# Autodesk Inventor assembly: buildplate
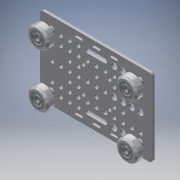
[picture p0: Inventor's stored thumbnail of the model, 180x180]
Saved by Autodesk Inventor 2016 (Build 200138000, 138)
## iProperties
Created: 2016-03-19
Part Number: buildplate
Document SubType Name: Assembly
Designer: Solomon
Author: Solomon
## Documents named in this file (4)
- C:\Users\Solomon\Documents\Inventor\SLA MK I\buildplate.iam
- C:\Users\Solomon\Documents\Inventor\SLA MK I\V Slot Part Files\V Slot Plates\Large Build Plate.ipt
- C:\Users\Solomon\Documents\Inventor\SLA MK I\vwheel.iam
- C:\Users\Solomon\Documents\Inventor\SLA MK I\V Slot Part Files\Spacers\Normal M5 Wheel Spacer.ipt
## Components (9 placed, 3 different names)
1. Large Build Plate:1 — Mate:5, Mate:6, Mate:7, Mate:8
2. vwheel:1 [sub-assembly] — Mate:1, Angle:1
3. Normal M5 Wheel Spacer:1 — Mate:1, Angle:1, Mate:5
4. vwheel:2 [sub-assembly]
5. Normal M5 Wheel Spacer:2 — Mate:6
6. vwheel:3 [sub-assembly]
7. Normal M5 Wheel Spacer:3 — Mate:8
8. vwheel:4 [sub-assembly]
9. Normal M5 Wheel Spacer:4 — Mate:7
## Relationships (12: Mate 8, Angle 4)
- Mate:1: vwheel:1 ↔ Normal M5 Wheel Spacer:1
- Angle:1 (0 deg): vwheel:1 ↔ Normal M5 Wheel Spacer:1
- [Mate]: vwheel:2 ↔ Normal M5 Wheel Spacer:2
- [Angle] (0 deg): vwheel:2 ↔ Normal M5 Wheel Spacer:2
- [Mate]: vwheel:3 ↔ Normal M5 Wheel Spacer:3
- [Angle] (0 deg): vwheel:3 ↔ Normal M5 Wheel Spacer:3
- [Mate]: vwheel:4 ↔ Normal M5 Wheel Spacer:4
- [Angle] (0 deg): vwheel:4 ↔ Normal M5 Wheel Spacer:4
- Mate:5: Large Build Plate:1 ↔ Normal M5 Wheel Spacer:1
- Mate:6: Large Build Plate:1 ↔ Normal M5 Wheel Spacer:2
- Mate:7: Large Build Plate:1 ↔ Normal M5 Wheel Spacer:4
- Mate:8: Large Build Plate:1 ↔ Normal M5 Wheel Spacer:3
## Named parameters: d2_d0 = 0 mm, d3_d1 = 0 deg, d4_d0 = 0 mm, d5_d1 = 0 deg, d6_d0 = 0 mm, d7_d1 = 0 deg
